# Autodesk Inventor assembly: TurretAssembly
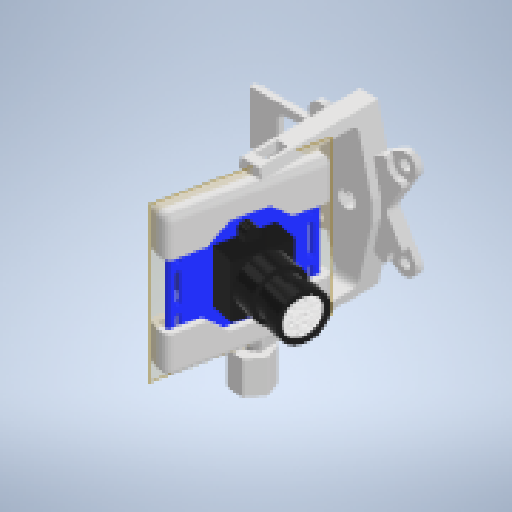
[picture p0: Inventor's stored thumbnail of the model, 512x512]
Saved by Autodesk Inventor 2023 (Build 270158000, 158)
## iProperties
Created: 2023-05-07
Part Number: TurretAssembly
Document SubType Name: Assembly
Designer: karpova
Author: karpova
## Documents named in this file (6)
- C:\_dev\24-transcription-study-assistant\cad-files\SeniorDesign_V0\TurretAssembly.iam
- C:\_dev\24-transcription-study-assistant\cad-files\SeniorDesign_V0\TurretBase.ipt
- C:\_dev\24-transcription-study-assistant\cad-files\SeniorDesign_V0\TurretPressFit.ipt
- C:\_dev\24-transcription-study-assistant\cad-files\SeniorDesign_V0\Camera2.ipt
- C:\_dev\24-transcription-study-assistant\cad-files\SeniorDesign_V0\TurretCameraCover.ipt
- C:\_dev\24-transcription-study-assistant\cad-files\SeniorDesign_V0\TurretTighteningNut.ipt
## Components (5 placed, 5 different names)
1. TurretBase:1
2. TurretPressFit:1 — Mate:1, Mate:3, Mate:4, Mate:5
3. Camera2:1 — Flush:2
4. TurretCameraCover:1 — Flush:2, Mate:1, Mate:4, Mate:5
5. TurretTighteningNut:1 — Mate:3
## Relationships (5: Mate 4, Flush 1)
- Flush:2: Camera2:1 ↔ TurretCameraCover:1
- Mate:1: TurretPressFit:1 ↔ TurretCameraCover:1
- Mate:3: TurretPressFit:1 ↔ TurretTighteningNut:1
- Mate:4: TurretPressFit:1 ↔ TurretCameraCover:1
- Mate:5: TurretPressFit:1 ↔ TurretCameraCover:1
